# Autodesk Inventor assembly: EnsamblajeCajaElectricaCompletaV2
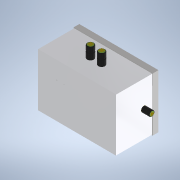
[picture p0: Inventor's stored thumbnail of the model, 180x180]
Saved by Autodesk Inventor 2020 (Build 240168000, 168)
## iProperties
Created: 2021-12-16
Part Number: EnsamblajeCajaElectricaCompletaV2
Document SubType Name: Assembly
Designer: DANIEL
Mass: 892.08 g
Surface Area: 3806.95 cm^2
Volume: 892.08 cm^3
Density: 1 g/cm^3
Author: DANIEL
## Documents named in this file (9)
- C:\Users\DANIEL\Documents\Personal\Convocatorias\Escollera\tesis\CAD\V3\EnsamblajeCajaElectricaCompletaV3.iam
- C:\Users\DANIEL\Documents\Personal\Convocatorias\Escollera\tesis\CAD\V3\EnsamblajeCircuito.iam
- C:\Users\DANIEL\Documents\Personal\Convocatorias\Escollera\tesis\CAD\V3\CARGADOR BATERIA LIPO LITIO 4 CELDAS 5A 18650.ipt
- C:\Users\DANIEL\Documents\Personal\Convocatorias\Escollera\tesis\CAD\V3\cajaEléctrica.ipt
- C:\Users\DANIEL\Documents\Personal\Convocatorias\Escollera\tesis\CAD\V3\portabateriasConBaterias.iam
- C:\Users\DANIEL\Documents\Personal\Convocatorias\Escollera\tesis\CAD\V3\unionImpermeableDe2o3pines.ipt
- C:\Users\DANIEL\Documents\Personal\Convocatorias\Escollera\tesis\CAD\V3\unionImpermeableDe4pines.ipt
- C:\Users\DANIEL\Documents\Personal\Convocatorias\Escollera\tesis\CAD\V3\antenaCodo.ipt
- C:\Users\DANIEL\Documents\Personal\Convocatorias\Escollera\tesis\CAD\V3\EnsamblajeCajaElectricaCompletaV3\AIP\Tubos y tuberías\Cable y arnés\EnsamblajeCajaElectricaCompletaV3.Arnés1.iam
## Components (9 placed, 8 different names)
1. EnsamblajeCircuito:1 [sub-assembly] — Coincidencia:3
2. CARGADOR BATERIA LIPO LITIO 4 CELDAS 5A 18650:1 — Coincidencia:2
3. cajaEléctrica:1 — Coincidencia:2, Coincidencia:3, Rígido:2, Rígido:3, Rígido:4, Plana:1, Coincidencia:5, Rígido:5
4. portabateriasConBaterias:1 [sub-assembly] — Plana:1
5. unionImpermeableDe2o3pines:1 — Rígido:3
6. unionImpermeableDe4pines:1 — Rígido:4
7. unionImpermeableDe4pines:2 — Rígido:2
8. antenaCodo:1 — Rígido:5
9. Arnés1 [sub-assembly]
## Relationships (8: WeldJoint 4, Mate 3, PlanarJoint 1)
- Coincidencia:2 [Mate]: CARGADOR BATERIA LIPO LITIO 4 CELDAS 5A 18650:1 ↔ cajaEléctrica:1
- Coincidencia:3 [Mate]: EnsamblajeCircuito:1 ↔ cajaEléctrica:1
- Rígido:2 [WeldJoint] (3.5 mm): cajaEléctrica:1 ↔ unionImpermeableDe4pines:2
- Rígido:3 [WeldJoint] (1.5 mm): cajaEléctrica:1 ↔ unionImpermeableDe2o3pines:1
- Rígido:4 [WeldJoint]: cajaEléctrica:1 ↔ unionImpermeableDe4pines:1
- Plana:1: cajaEléctrica:1 ↔ portabateriasConBaterias:1
- Coincidencia:5 [Mate]: cajaEléctrica:1
- Rígido:5 [WeldJoint]: cajaEléctrica:1 ↔ antenaCodo:1
